# Autodesk Inventor assembly: Rr.wing(flap4)_cradle
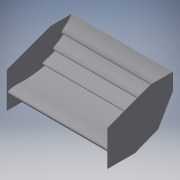
[picture p0: Inventor's stored thumbnail of the model, 180x180]
Saved by Autodesk Inventor 2018.2 (Build 222227000, 227)
## iProperties
Created: 2018-03-07
Part Number: Rr.wing(flap4)_cradle
Material: 一般
Document SubType Name: Assembly
Designer: ku_sk
Author: ku_sk
## Documents named in this file (4)
- C:\Users\ku_sk\Documents\Inventor\Aero\KS-15\Rr.wing\cradle\base_model\Rr.wing_cradle\Rr.wing(flap4)_cradle.iam
- C:\Users\ku_sk\Documents\Inventor\Aero\KS-15\Rr.wing\cradle\base_model\Rr.wing_cradle\parts\main frap.ipt
- C:\Users\ku_sk\Documents\Inventor\Aero\KS-15\Rr.wing\cradle\base_model\Rr.wing_cradle\parts\subflap.ipt
- C:\Users\ku_sk\Documents\Inventor\Aero\KS-15\Rr.wing\cradle\base_model\Rr.wing_cradle\parts\endplate(flap4).ipt
## Components (6 placed, 3 different names)
1. main frap:1 — メイト:1, フラッシュ:1, メイト:2, メイト:3, 角度:1, メイト:7, メイト:8, 角度:2
2. subflap:1 — メイト:4, 角度:2, 角度:3, メイト:9
3. subflap:2 — メイト:5, 角度:3, 角度:4, メイト:10
4. subflap:3 — メイト:6, 角度:4, メイト:11
5. endplate(flap4):1 — メイト:2, メイト:7, フラッシュ:2, フラッシュ:3, 角度:5
6. endplate(flap4):2 — メイト:3, メイト:4, メイト:5, メイト:6, メイト:8, メイト:9, メイト:10, メイト:11, フラッシュ:2, フラッシュ:3
## Relationships (19: Mate 11, Angle 5, Flush 3)
- メイト:1 [Mate]: main frap:1
- フラッシュ:1 [Flush]: main frap:1
- メイト:2 [Mate]: main frap:1 ↔ endplate(flap4):1
- メイト:3 [Mate]: main frap:1 ↔ endplate(flap4):2
- メイト:4 [Mate]: subflap:1 ↔ endplate(flap4):2
- メイト:5 [Mate]: subflap:2 ↔ endplate(flap4):2
- メイト:6 [Mate]: subflap:3 ↔ endplate(flap4):2
- 角度:1 [Angle] (-15 deg): main frap:1
- メイト:7 [Mate]: main frap:1 ↔ endplate(flap4):1
- メイト:8 [Mate]: main frap:1 ↔ endplate(flap4):2
- 角度:2 [Angle] (15 deg): main frap:1 ↔ subflap:1
- 角度:3 [Angle] (-15 deg): subflap:1 ↔ subflap:2
- 角度:4 [Angle] (10 deg): subflap:2 ↔ subflap:3
- メイト:9 [Mate]: subflap:1 ↔ endplate(flap4):2
- メイト:10 [Mate]: subflap:2 ↔ endplate(flap4):2
- メイト:11 [Mate]: subflap:3 ↔ endplate(flap4):2
- フラッシュ:2 [Flush]: endplate(flap4):1 ↔ endplate(flap4):2
- フラッシュ:3 [Flush]: endplate(flap4):1 ↔ endplate(flap4):2
- 角度:5 [Angle] (0 deg): endplate(flap4):1
